# Autodesk Inventor assembly: Assembly1
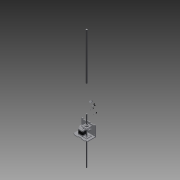
[picture p0: Inventor's stored thumbnail of the model, 180x180]
Saved by Autodesk Inventor 2015 (Build 190159000, 159)
## iProperties
Created: 2017-03-07
Part Number: Assembly1
Document SubType Name: Assembly
Designer: Ernest
Author: Ernest
## Documents named in this file (17)
- C:\Users\Ernest\Documents\Capstone-Project\doc\CAD\EndEffectorBase2\Assembly1.iam
- C:\Users\Ernest\Documents\Capstone-Project\doc\CAD\EndEffectorBase2\ThreadBar90.ipt
- C:\Users\Ernest\Documents\Capstone-Project\doc\CAD\EndEffectorBase2\ThreadBar127.ipt
- C:\Users\Ernest\Documents\Capstone-Project\doc\CAD\Stepper Motor\NEMA-17\NEMA 17.iam
- C:\Users\Ernest\Documents\Capstone-Project\doc\CAD\Gears\Spur Gears1.iam
- C:\Users\Ernest\Documents\Capstone-Project\doc\CAD\Sensors\LineSensor.ipt
- C:\Users\Ernest\Documents\Capstone-Project\doc\CAD\Sensors\LinesensorHolderBottom.ipt
- C:\Users\Ernest\Documents\Capstone-Project\doc\CAD\Sensors\LinesensorHolderTop.ipt
- C:\Users\Ernest\Documents\Capstone-Project\doc\CAD\Sensors\LinesensorHolderWasher.ipt
- C:\Users\Ernest\Documents\Capstone-Project\doc\CAD\EndEffectorBase2\BigPositionDisk.ipt
- C:\Users\Ernest\Documents\Capstone-Project\doc\CAD\EndEffectorBase2\SmallPositionDisk.ipt
- C:\Users\Ernest\Documents\Capstone-Project\doc\CAD\LowLevel_Rev3\EE_base\EE_base_assembly.iam
- C:\Users\Ernest\Documents\Capstone-Project\doc\CAD\EndEffectorBase2\BallBearing.ipt
- C:\Users\Ernest\Documents\Capstone-Project\doc\CAD\EndEffectorBase2\BallBearingCenterer.ipt
- C:\Users\Ernest\Documents\Capstone-Project\doc\CAD\EndEffectorBase2\9mmRodNut.ipt
- C:\Users\Ernest\Documents\Capstone-Project\doc\CAD\EndEffectorBase2\BallBearingHolderTop.ipt
- C:\Users\Ernest\Documents\Capstone-Project\doc\CAD\EndEffectorBase2\BallBearingHolderBottom.ipt
## Components (27 placed, 16 different names)
1. ThreadBar90:1 — Mate:14, Mate:15, Mate:22, Mate:23, Mate:24, Mate:25, Mate:31
2. ThreadBar127:1 — Mate:15
3. NEMA 17:1 [sub-assembly] — Mate:1, Mate:26, Angle:1, Mate:32
4. Spur Gears:1 [sub-assembly] — Mate:1, Mate:14, Mate:16, Mate:17, Mate:18, Mate:28, Mate:30
5. LineSensor:1
6. LineSensor:2
7. LineSensor:3
8. LineSensor:4
9. LinesensorHolderBottom:1 — Mate:9, Mate:10, Mate:11, Mate:12, Mate:13
10. LinesensorHolderBottom:2 — Mate:5, Mate:6, Mate:7
11. LinesensorHolderTop:1 — Mate:8, Mate:12, Mate:13
12. LinesensorHolderTop:2 — Mate:2, Mate:3, Mate:4, Mate:5, Mate:7
13. LinesensorHolderWasher:1 — Mate:2, Mate:3, Mate:4, Mate:6
14. LinesensorHolderWasher:2 — Mate:8, Mate:9, Mate:10, Mate:11
15. BigPositionDisk:1 — Mate:31
16. SmallPositionDisk:1 — Mate:32
17. EE_base_assembly:1 [sub-assembly] — Mate:18, Flush:1, Angle:1, Angle:2, Mate:29, Angle:3
18. BallBearing:1 — Mate:16, Mate:19, Mate:20, Flush:3, Mate:27
19. BallBearing:2 — Mate:17, Mate:19, Flush:1, Mate:21, Flush:2, Mate:26
20. BallBearingCenterer:1 — Mate:20, Flush:3
21. BallBearingCenterer:2 — Mate:21, Flush:2
22. 9mmRodNut:1 — Mate:24
23. 9mmRodNut:2 — Mate:25
24. 9mmRodNut:3 — Mate:22
25. 9mmRodNut:4 — Mate:23
26. BallBearingHolderTop:1 — Mate:27, Mate:28, Angle:2
27. BallBearingHolderBottom:1 — Mate:29, Mate:30, Angle:3
## Relationships (38: Mate 32, Flush 3, Angle 3)
- Mate:1: NEMA 17:1 ↔ Spur Gears:1
- Mate:2: LinesensorHolderTop:2 ↔ LinesensorHolderWasher:1
- Mate:3: LinesensorHolderTop:2 ↔ LinesensorHolderWasher:1
- Mate:4: LinesensorHolderTop:2 ↔ LinesensorHolderWasher:1
- Mate:5: LinesensorHolderBottom:2 ↔ LinesensorHolderTop:2
- Mate:6: LinesensorHolderBottom:2 ↔ LinesensorHolderWasher:1
- Mate:7: LinesensorHolderBottom:2 ↔ LinesensorHolderTop:2
- Mate:8: LinesensorHolderTop:1 ↔ LinesensorHolderWasher:2
- Mate:9: LinesensorHolderBottom:1 ↔ LinesensorHolderWasher:2
- Mate:10: LinesensorHolderBottom:1 ↔ LinesensorHolderWasher:2
- Mate:11: LinesensorHolderBottom:1 ↔ LinesensorHolderWasher:2
- Mate:12: LinesensorHolderBottom:1 ↔ LinesensorHolderTop:1
- Mate:13: LinesensorHolderBottom:1 ↔ LinesensorHolderTop:1
- Mate:14: ThreadBar90:1 ↔ Spur Gears:1
- Mate:15: ThreadBar90:1 ↔ ThreadBar127:1
- Mate:16: Spur Gears:1 ↔ BallBearing:1
- Mate:17: Spur Gears:1 ↔ BallBearing:2
- Mate:18: Spur Gears:1 ↔ EE_base_assembly:1
- Mate:19 (78.125 mm): BallBearing:1 ↔ BallBearing:2
- Flush:1: EE_base_assembly:1 ↔ BallBearing:2
- Mate:20: BallBearing:1 ↔ BallBearingCenterer:1
- Mate:21: BallBearing:2 ↔ BallBearingCenterer:2
- Flush:2 (0.4 mm): BallBearing:2 ↔ BallBearingCenterer:2
- Flush:3 (0.4 mm): BallBearing:1 ↔ BallBearingCenterer:1
- Mate:22: ThreadBar90:1 ↔ 9mmRodNut:3
- Mate:23: ThreadBar90:1 ↔ 9mmRodNut:4
- Mate:24: ThreadBar90:1 ↔ 9mmRodNut:1
- Mate:25: ThreadBar90:1 ↔ 9mmRodNut:2
- Mate:26 (4 mm): NEMA 17:1 ↔ BallBearing:2
- Angle:1 (0 deg): NEMA 17:1 ↔ EE_base_assembly:1
- Mate:27: BallBearing:1 ↔ BallBearingHolderTop:1
- Mate:28: Spur Gears:1 ↔ BallBearingHolderTop:1
- Angle:2 (0 deg): EE_base_assembly:1 ↔ BallBearingHolderTop:1
- Mate:29: EE_base_assembly:1 ↔ BallBearingHolderBottom:1
- Mate:30: Spur Gears:1 ↔ BallBearingHolderBottom:1
- Angle:3 (0 deg): EE_base_assembly:1 ↔ BallBearingHolderBottom:1
- Mate:31: ThreadBar90:1 ↔ BigPositionDisk:1
- Mate:32: NEMA 17:1 ↔ SmallPositionDisk:1
